# Autodesk Inventor assembly: Darrieus Turbine Assy
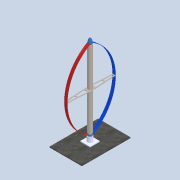
[picture p0: Inventor's stored thumbnail of the model, 180x180]
Saved by Autodesk Inventor 2020 (Build 240168000, 168)
## iProperties
Created: 2012-03-26
Part Number: Darrieus Turbine Assy
Description: STEP AP214
Document SubType Name: Assembly
Designer: Mathieu
Sending System: SolidWorks 2012
Preprocessor: SwSTEP 2.0
Title: Darrieus Turbine Assy.STEP
Author: 4745G
Revision Number: ANY
## Documents named in this file (5)
- C:\Users\Mathieu\switchdrive\HEVs\03-Cours\243-Elements de machines-DM-S4\Semestre 4\Exercices\Vis assemblage\TutorialInventorAssemblageVis\VisAssemblage-Tutoriel-FixationEolienne\Darrieus Turbine Assy.iam
- C:\Users\Mathieu\switchdrive\HEVs\03-Cours\243-Elements de machines-DM-S4\Semestre 4\Exercices\Vis assemblage\TutorialInventorAssemblageVis\VisAssemblage-Tutoriel-FixationEolienne\Mat.ipt
- C:\Users\Mathieu\switchdrive\HEVs\03-Cours\243-Elements de machines-DM-S4\Semestre 4\Exercices\Vis assemblage\TutorialInventorAssemblageVis\VisAssemblage-Tutoriel-FixationEolienne\Airfoil Darieus NACA 63-212.ipt
- C:\Users\Mathieu\switchdrive\HEVs\03-Cours\243-Elements de machines-DM-S4\Semestre 4\Exercices\Vis assemblage\TutorialInventorAssemblageVis\VisAssemblage-Tutoriel-FixationEolienne\Pied.ipt
- C:\Users\Mathieu\switchdrive\HEVs\03-Cours\243-Elements de machines-DM-S4\Semestre 4\Exercices\Vis assemblage\TutorialInventorAssemblageVis\VisAssemblage-Tutoriel-FixationEolienne\PlaqueSupport.ipt
## Components (4 placed, 4 different names)
1. Pied — Mate:1, Mate:2, Mate:3, Mate:4, Mate:5
2. Mat — Mate:6, Mate:7
3. Airfoil Darieus NACA 63-212_2 — Mate:4, Mate:5, Mate:6, Mate:7
4. PlaqueSupport:1 — Mate:1, Mate:2, Mate:3
## Relationships (7: Mate 7)
- Mate:1: Pied ↔ PlaqueSupport:1
- Mate:2: Pied ↔ PlaqueSupport:1
- Mate:3: Pied ↔ PlaqueSupport:1
- Mate:4: Pied ↔ Airfoil Darieus NACA 63-212_2
- Mate:5: Pied ↔ Airfoil Darieus NACA 63-212_2
- Mate:6: Mat ↔ Airfoil Darieus NACA 63-212_2
- Mate:7: Mat ↔ Airfoil Darieus NACA 63-212_2
